# Autodesk Inventor assembly: wheel slider assembely
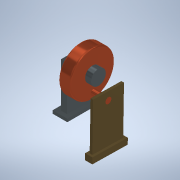
[picture p0: Inventor's stored thumbnail of the model, 180x180]
Saved by Autodesk Inventor 2021 (Build 250183000, 183)
## iProperties
Created: 2021-07-14
Part Number: wheel slider assembely
Document SubType Name: Assembly
Designer: Asus
Author: Asus
## Documents named in this file (4)
- E:\virtual\Wheel slider 1.2\wheel slider assembely.iam
- E:\virtual\Wheel slider 1.2\base stand.ipt
- E:\virtual\Wheel slider 1.2\wheel 1.2.ipt
- E:\virtual\Wheel slider 1.2\T-shape 1.3.ipt
## Components (3 placed, 3 different names)
1. base stand:1 — Mate:1, Mate:2
2. wheel 1.2:1 — Mate:1, Mate:2, Mate:3, Mate:4
3. T-shape 1.3:1 — Mate:3, Mate:4
## Relationships (4: Mate 4)
- Mate:1: base stand:1 ↔ wheel 1.2:1
- Mate:2: base stand:1 ↔ wheel 1.2:1
- Mate:3: wheel 1.2:1 ↔ T-shape 1.3:1
- Mate:4: wheel 1.2:1 ↔ T-shape 1.3:1
